# Autodesk Inventor assembly: door assembly
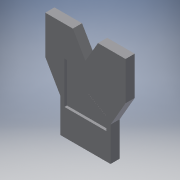
[picture p0: Inventor's stored thumbnail of the model, 180x180]
Saved by Autodesk Inventor 2017 (Build 210142000, 142)
## iProperties
Created: 2018-03-29
Part Number: door assembly
Document SubType Name: Assembly
Designer: braxtonwright
Author: braxtonwright
## Documents named in this file (7)
- D:\School\Game develpment\geoscape\done\doors\end door\9 foot door\door assembly.iam
- D:\School\Game develpment\geoscape\done\doors\end door\9 foot door\end door frame.ipt
- D:\School\Game develpment\geoscape\done\doors\end door\9 foot door\top left door.ipt
- D:\School\Game develpment\geoscape\done\doors\end door\9 foot door\top right door.ipt
- D:\School\Game develpment\geoscape\done\doors\end door\9 foot door\bottom door.ipt
- D:\School\Game develpment\geoscape\done\doors\end door\9 foot door\left and right hiding bar.ipt
- D:\School\Game develpment\geoscape\done\doors\end door\9 foot door\bottom and top hiding bar.ipt
## Components (12 placed, 6 different names)
1. end door frame:1 — Mate:1, Mate:2, Mate:3, Mate:4, Mate:5, Mate:6, Mate:7, Mate:8, Mate:11, Mate:12, Mate:13, Mate:14, Mate:15, Mate:16, Mate:17, Mate:18, Mate:19, Mate:20, Mate:21, Mate:22, Mate:23, Mate:24, Mate:25, Mate:26, Mate:27, Mate:28, Mate:29, Mate:30, Mate:31, Mate:32, Mate:33, Mate:34
2. top left door:1 — Mate:1, Mate:2, Mate:3, Mate:10
3. top right door:1 — Mate:4, Mate:5, Mate:6, Mate:9
4. bottom door:1 — Mate:7, Mate:8, Mate:9, Mate:10
5. left and right hiding bar:1 — Mate:26, Mate:30, Mate:31
6. left and right hiding bar:2 — Mate:17, Mate:19, Mate:21
7. left and right hiding bar:3 — Mate:18, Mate:20, Mate:22
8. left and right hiding bar:4 — Mate:25, Mate:29, Mate:32
9. bottom and top hiding bar:1 — Mate:11, Mate:13, Mate:16
10. bottom and top hiding bar:2 — Mate:12, Mate:14, Mate:15
11. bottom and top hiding bar:3 — Mate:24, Mate:28, Mate:33
12. bottom and top hiding bar:4 — Mate:23, Mate:27, Mate:34
## Relationships (34: Mate 34)
- Mate:1: end door frame:1 ↔ top left door:1
- Mate:2: end door frame:1 ↔ top left door:1
- Mate:3: end door frame:1 ↔ top left door:1
- Mate:4: end door frame:1 ↔ top right door:1
- Mate:5: end door frame:1 ↔ top right door:1
- Mate:6: end door frame:1 ↔ top right door:1
- Mate:7: end door frame:1 ↔ bottom door:1
- Mate:8: end door frame:1 ↔ bottom door:1
- Mate:9: top right door:1 ↔ bottom door:1
- Mate:10: top left door:1 ↔ bottom door:1
- Mate:11: end door frame:1 ↔ bottom and top hiding bar:1
- Mate:12: end door frame:1 ↔ bottom and top hiding bar:2
- Mate:13: end door frame:1 ↔ bottom and top hiding bar:1
- Mate:14: end door frame:1 ↔ bottom and top hiding bar:2
- Mate:15: end door frame:1 ↔ bottom and top hiding bar:2
- Mate:16: end door frame:1 ↔ bottom and top hiding bar:1
- Mate:17: end door frame:1 ↔ left and right hiding bar:2
- Mate:18: end door frame:1 ↔ left and right hiding bar:3
- Mate:19: end door frame:1 ↔ left and right hiding bar:2
- Mate:20: end door frame:1 ↔ left and right hiding bar:3
- Mate:21: end door frame:1 ↔ left and right hiding bar:2
- Mate:22: end door frame:1 ↔ left and right hiding bar:3
- Mate:23: end door frame:1 ↔ bottom and top hiding bar:4
- Mate:24: end door frame:1 ↔ bottom and top hiding bar:3
- Mate:25: end door frame:1 ↔ left and right hiding bar:4
- Mate:26: end door frame:1 ↔ left and right hiding bar:1
- Mate:27: end door frame:1 ↔ bottom and top hiding bar:4
- Mate:28: end door frame:1 ↔ bottom and top hiding bar:3
- Mate:29: end door frame:1 ↔ left and right hiding bar:4
- Mate:30: end door frame:1 ↔ left and right hiding bar:1
- Mate:31: end door frame:1 ↔ left and right hiding bar:1
- Mate:32: end door frame:1 ↔ left and right hiding bar:4
- Mate:33: end door frame:1 ↔ bottom and top hiding bar:3
- Mate:34: end door frame:1 ↔ bottom and top hiding bar:4
